# Autodesk Inventor assembly: 5th Wheel Hitch Fix
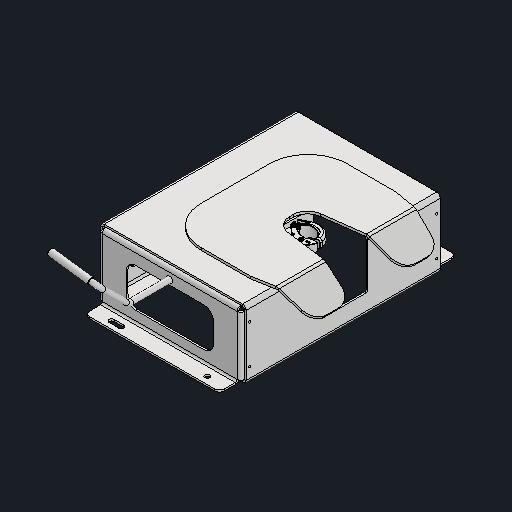
[picture p0: Inventor's stored thumbnail of the model, 512x512]
Saved by Autodesk Inventor 2025.1 (Build 291241000, 241)
## iProperties
Created: 2026-02-24
Part Number: 5th Wheel Hitch Fix
Document SubType Name: Assembly
Designer: Desktop -24
Author: Desktop -24
## Documents named in this file (6)
- F:\OneDrive - nLeague Technologies Private Limited\Desktop\Sharath Chandra\5th Wheel Hitch\5th Wheel Hitch Fix.iam
- F:\OneDrive - nLeague Technologies Private Limited\Desktop\Sharath Chandra\5th Wheel Hitch\5th Wheel Hitch Part 1.ipt
- F:\OneDrive - nLeague Technologies Private Limited\Desktop\Sharath Chandra\5th Wheel Hitch\5th Wheel Hitch Part 2.ipt
- F:\OneDrive - nLeague Technologies Private Limited\Desktop\Sharath Chandra\5th Wheel Hitch\5th Wheel Hitch Part 3.ipt
- F:\OneDrive - nLeague Technologies Private Limited\Desktop\Sharath Chandra\5th Wheel Hitch\5th Wheel Hitch Part 4.ipt
- F:\OneDrive - nLeague Technologies Private Limited\Desktop\Sharath Chandra\5th Wheel Hitch\5th Wheel Hitch Part 5.ipt
## Components (6 placed, 5 different names)
1. 5th Wheel Hitch Part 1:1 — Mate:1, Mate:2, Flush:1, Flush:2, Flush:3, Flush:4, Mate:3, Mate:4, Mate:5, Mate:6, Mate:7, Mate:8, Mate:9, Mate:11, Flush:5
2. 5th Wheel Hitch Part 2:1 — Mate:2, Flush:4, Mate:3, Flush:6
3. 5th Wheel Hitch Part 3:1 — Mate:4, Mate:6, Mate:8, Mate:10
4. 5th Wheel Hitch Part 3:2 — Mate:5, Mate:7, Mate:9
5. 5th Wheel Hitch Part 4:1 — Mate:10
6. 5th Wheel Hitch Part 5:1 — Mate:11, Flush:5, Flush:6
## Relationships (17: Mate 11, Flush 6)
- Mate:1: 5th Wheel Hitch Part 1:1
- Mate:2: 5th Wheel Hitch Part 1:1 ↔ 5th Wheel Hitch Part 2:1
- Flush:1: 5th Wheel Hitch Part 1:1
- Flush:2: 5th Wheel Hitch Part 1:1
- Flush:3: 5th Wheel Hitch Part 1:1
- Flush:4: 5th Wheel Hitch Part 1:1 ↔ 5th Wheel Hitch Part 2:1
- Mate:3: 5th Wheel Hitch Part 1:1 ↔ 5th Wheel Hitch Part 2:1
- Mate:4: 5th Wheel Hitch Part 1:1 ↔ 5th Wheel Hitch Part 3:1
- Mate:5: 5th Wheel Hitch Part 1:1 ↔ 5th Wheel Hitch Part 3:2
- Mate:6: 5th Wheel Hitch Part 1:1 ↔ 5th Wheel Hitch Part 3:1
- Mate:7: 5th Wheel Hitch Part 1:1 ↔ 5th Wheel Hitch Part 3:2
- Mate:8: 5th Wheel Hitch Part 1:1 ↔ 5th Wheel Hitch Part 3:1
- Mate:9: 5th Wheel Hitch Part 1:1 ↔ 5th Wheel Hitch Part 3:2
- Mate:10: 5th Wheel Hitch Part 3:1 ↔ 5th Wheel Hitch Part 4:1
- Mate:11: 5th Wheel Hitch Part 1:1 ↔ 5th Wheel Hitch Part 5:1
- Flush:5: 5th Wheel Hitch Part 1:1 ↔ 5th Wheel Hitch Part 5:1
- Flush:6: 5th Wheel Hitch Part 2:1 ↔ 5th Wheel Hitch Part 5:1
